# Autodesk Inventor assembly: WristAssembly
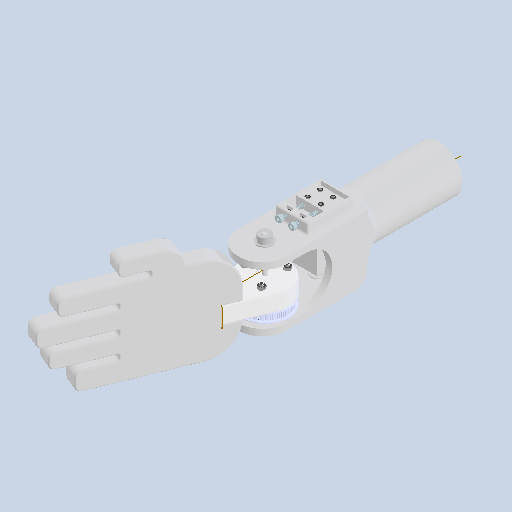
[picture p0: Inventor's stored thumbnail of the model, 512x512]
Saved by Autodesk Inventor 2024 (Build 280153000, 153)
## iProperties
Created: 2024-02-05
Part Number: WristAssembly
Document SubType Name: Assembly
Designer: Irwin
Author: Irwin
## Documents named in this file (18)
- C:\Users\anyangoe\Desktop\WholeRobot\WristAssembly.iam
- WristAssembly.iam
- C:\Users\anyangoe\Desktop\WholeRobot\WristConnect.ipt
- C:\Users\anyangoe\Desktop\WholeRobot\F625ZZ Ball Bearing.ipt
- C:\Users\anyangoe\Desktop\WholeRobot\5mmShaft.ipt
- C:\Users\anyangoe\Desktop\WholeRobot\AS 1420 - 1973 - M3 x 20.ipt
- C:\Users\anyangoe\Desktop\WholeRobot\GT2 5MM 80T.ipt
- C:\Users\anyangoe\Desktop\WholeRobot\Lock Collar 5mm.ipt
- C:\Users\anyangoe\Desktop\WholeRobot\WristMotor.ipt
- C:\Users\anyangoe\Desktop\WholeRobot\GT2_20T.ipt
- C:\Users\anyangoe\Desktop\WholeRobot\WristMotorTensioner.ipt
- C:\Users\anyangoe\Desktop\WholeRobot\M4x25.ipt
- C:\Users\anyangoe\Desktop\WholeRobot\PulleytoHand.ipt
- C:\Users\anyangoe\Desktop\WholeRobot\Handv3.ipt
- C:\Users\anyangoe\Desktop\WholeRobot\AS 1427 - M4 x 35(5) II.ipt
- C:\Users\anyangoe\Desktop\WholeRobot\AS 1112 - M4  Type 8.ipt
- C:\Users\anyangoe\Desktop\WholeRobot\AS 1427 - M3 x 40(5) II.ipt
- C:\Users\anyangoe\Desktop\WholeRobot\AS 1112 - M3  Type 8.ipt
## Components (30 placed, 16 different names)
1. WristConnect:1 — Mate:1, Mate:2, Mate:3, Mate:4, Flush:1, Mate:31, Angle:1, Mate:34, Flush:6, Mate:35, Mate:36, Mate:75, Mate:76
2. F625ZZ Ball Bearing:1 — Mate:1, Mate:2, Mate:25
3. F625ZZ Ball Bearing:2 — Mate:3, Mate:4, Mate:5, Mate:23
4. 5mmShaft:1 — Mate:5, Flush:1, Mate:22, Mate:24, Mate:47, Mate:48
5. GT2 5MM 80T:1 — Mate:48, Flush:7, Mate:53, Mate:54, Mate:58, Mate:59, Mate:60
6. Lock Collar 5mm:1 — Mate:22, Mate:23
7. Lock Collar 5mm:2 — Mate:24, Mate:25
8. WristMotor:1 — Mate:31, Angle:1, Mate:32, Mate:33
9. GT2_20T:1 — Mate:32, Mate:33, Flush:7
10. WristMotorTensioner:1 — Mate:34, Flush:6, Mate:37, Mate:38, Mate:39, Mate:40, Mate:41, Mate:42, Mate:43, Mate:44, Mate:45, Mate:46
11. M4x25:1 — Mate:35, Mate:37, Mate:73
12. M4x25:2 — Mate:36, Mate:38, Mate:74
13. AS 1420 - Metric M3 x 20:1 — Mate:39, Mate:43
14. AS 1420 - Metric M3 x 20:2 — Mate:42, Mate:45
15. AS 1420 - Metric M3 x 20:3 — Mate:41, Mate:44
16. AS 1420 - Metric M3 x 20:4 — Mate:40, Mate:46
17. PulleytoHand:1 — Mate:47, Mate:50, Mate:51, Mate:52, Mate:53, Mate:54, Mate:55, Mate:56, Mate:57, Mate:64, Mate:65, Mate:66
18. Handv3:1 — Mate:50, Mate:51, Mate:52, Mate:67, Mate:68, Mate:69, Mate:70
19. AS 1427 H - Metric M4 x 35:1 — Mate:55, Mate:58, Mate:62
20. AS 1427 H - Metric M4 x 35:2 — Mate:56, Mate:59, Mate:61
21. AS 1427 H - Metric M4 x 35:3 — Mate:57, Mate:60, Mate:63
22. AS 1112 (2) - Metric M4  Type 8:1 — Mate:63, Mate:65
23. AS 1112 (2) - Metric M4  Type 8:2 — Mate:62, Mate:64
24. AS 1112 (2) - Metric M4  Type 8:3 — Mate:61, Mate:66
25. AS 1427 H - Metric M3 x 40:1 — Mate:67, Mate:70, Mate:71
26. AS 1427 H - Metric M3 x 40:2 — Mate:68, Mate:69, Mate:72
27. AS 1112 (2) - Metric M3  Type 8:1 — Mate:71
28. AS 1112 (2) - Metric M3  Type 8:2 — Mate:72
29. AS 1112 (2) - Metric M4  Type 8:4 — Mate:73, Mate:75
30. AS 1112 (2) - Metric M4  Type 8:5 — Mate:74, Mate:76
## Relationships (58: Mate 54, Flush 3, Angle 1)
- Mate:1: WristConnect:1 ↔ F625ZZ Ball Bearing:1
- Mate:2: WristConnect:1 ↔ F625ZZ Ball Bearing:1
- Mate:3: WristConnect:1 ↔ F625ZZ Ball Bearing:2
- Mate:4: WristConnect:1 ↔ F625ZZ Ball Bearing:2
- Mate:5: F625ZZ Ball Bearing:2 ↔ 5mmShaft:1
- Flush:1 (-8 mm): WristConnect:1 ↔ 5mmShaft:1
- Mate:22: 5mmShaft:1 ↔ Lock Collar 5mm:1
- Mate:23: F625ZZ Ball Bearing:2 ↔ Lock Collar 5mm:1
- Mate:24: 5mmShaft:1 ↔ Lock Collar 5mm:2
- Mate:25: F625ZZ Ball Bearing:1 ↔ Lock Collar 5mm:2
- Mate:31: WristConnect:1 ↔ WristMotor:1
- Angle:1 (0 deg): WristConnect:1 ↔ WristMotor:1
- Mate:32: WristMotor:1 ↔ GT2_20T:1
- Mate:33: WristMotor:1 ↔ GT2_20T:1
- Mate:34: WristConnect:1 ↔ WristMotorTensioner:1
- Flush:6: WristConnect:1 ↔ WristMotorTensioner:1
- Mate:35: WristConnect:1 ↔ M4x25:1
- Mate:36: WristConnect:1 ↔ M4x25:2
- Mate:37: WristMotorTensioner:1 ↔ M4x25:1
- Mate:38: WristMotorTensioner:1 ↔ M4x25:2
- Mate:39: WristMotorTensioner:1 ↔ AS 1420 - Metric M3 x 20:1
- Mate:40: WristMotorTensioner:1 ↔ AS 1420 - Metric M3 x 20:4
- Mate:41: WristMotorTensioner:1 ↔ AS 1420 - Metric M3 x 20:3
- Mate:42: WristMotorTensioner:1 ↔ AS 1420 - Metric M3 x 20:2
- Mate:43: WristMotorTensioner:1 ↔ AS 1420 - Metric M3 x 20:1
- Mate:44: WristMotorTensioner:1 ↔ AS 1420 - Metric M3 x 20:3
- Mate:45: WristMotorTensioner:1 ↔ AS 1420 - Metric M3 x 20:2
- Mate:46: WristMotorTensioner:1 ↔ AS 1420 - Metric M3 x 20:4
- Mate:47: 5mmShaft:1 ↔ PulleytoHand:1
- Mate:48: 5mmShaft:1 ↔ GT2 5MM 80T:1
- Flush:7: GT2 5MM 80T:1 ↔ GT2_20T:1
- Mate:50: PulleytoHand:1 ↔ Handv3:1
- Mate:51: PulleytoHand:1 ↔ Handv3:1
- Mate:52: PulleytoHand:1 ↔ Handv3:1
- Mate:53: GT2 5MM 80T:1 ↔ PulleytoHand:1
- Mate:54: GT2 5MM 80T:1 ↔ PulleytoHand:1
- Mate:55: PulleytoHand:1 ↔ AS 1427 H - Metric M4 x 35:1
- Mate:56: PulleytoHand:1 ↔ AS 1427 H - Metric M4 x 35:2
- Mate:57: PulleytoHand:1 ↔ AS 1427 H - Metric M4 x 35:3
- Mate:58: GT2 5MM 80T:1 ↔ AS 1427 H - Metric M4 x 35:1
- Mate:59: GT2 5MM 80T:1 ↔ AS 1427 H - Metric M4 x 35:2
- Mate:60: GT2 5MM 80T:1 ↔ AS 1427 H - Metric M4 x 35:3
- Mate:61: AS 1427 H - Metric M4 x 35:2 ↔ AS 1112 (2) - Metric M4  Type 8:3
- Mate:62: AS 1427 H - Metric M4 x 35:1 ↔ AS 1112 (2) - Metric M4  Type 8:2
- Mate:63: AS 1427 H - Metric M4 x 35:3 ↔ AS 1112 (2) - Metric M4  Type 8:1
- Mate:64: PulleytoHand:1 ↔ AS 1112 (2) - Metric M4  Type 8:2
- Mate:65: PulleytoHand:1 ↔ AS 1112 (2) - Metric M4  Type 8:1
- Mate:66: PulleytoHand:1 ↔ AS 1112 (2) - Metric M4  Type 8:3
- Mate:67: Handv3:1 ↔ AS 1427 H - Metric M3 x 40:1
- Mate:68: Handv3:1 ↔ AS 1427 H - Metric M3 x 40:2
- Mate:69: Handv3:1 ↔ AS 1427 H - Metric M3 x 40:2
- Mate:70: Handv3:1 ↔ AS 1427 H - Metric M3 x 40:1
- Mate:71: AS 1427 H - Metric M3 x 40:1 ↔ AS 1112 (2) - Metric M3  Type 8:1
- Mate:72: AS 1427 H - Metric M3 x 40:2 ↔ AS 1112 (2) - Metric M3  Type 8:2
- Mate:73: M4x25:1 ↔ AS 1112 (2) - Metric M4  Type 8:4
- Mate:74: M4x25:2 ↔ AS 1112 (2) - Metric M4  Type 8:5
- Mate:75: WristConnect:1 ↔ AS 1112 (2) - Metric M4  Type 8:4
- Mate:76: WristConnect:1 ↔ AS 1112 (2) - Metric M4  Type 8:5
